# Autodesk Inventor assembly: NT_BMP005_001_A_001
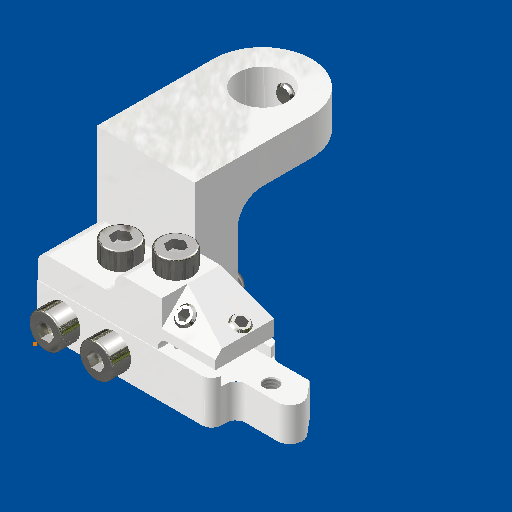
[picture p0: Inventor's stored thumbnail of the model, 512x512]
Saved by Autodesk Inventor 2025 (Build 290162000, 162)
## iProperties
Created: 2024-04-15
Part Number: NT_BMP005_001_A_001
Document SubType Name: Assembly
Designer: AdminForWorker
Mass: 69.6726 g
Surface Area: 73.8682 cm^2
Volume: 8.92251 cm^3
Density: 7.80863 g/cm^3
Title: NT_BMP005_001_A_001
Author: AdminForWorker
Revision Number: 1
## Documents named in this file (12)
- C:\Users\faricci\Inventor\Headframe_Edit\2_screws\Fabio_edit_2Screws.iam
- C:\Users\faricci\Inventor\Headframe_Edit\2_screws\Base.ipt
- C:\Users\faricci\Inventor\Headframe_Edit\2_screws\Top Base.ipt
- C:\Users\faricci\Inventor\Headframe_Edit\2_screws\Headpost_mirrored_2screws v5.ipt
- C:\Users\faricci\Inventor\Headframe_Edit\2_screws\Stereotaxic_mounting.ipt
- C:\Users\faricci\OneDrive - Fondazione Istituto Italiano Tecnologia\Documents\Inventor\Content Center Files\R2025\en-US\ISO 4026\ISO 4026 - M3 x 5 - ISO.ipt
- C:\Users\faricci\OneDrive - Fondazione Istituto Italiano Tecnologia\Documents\Inventor\Content Center Files\R2025\en-US\ISO 4026\ISO 4026 - M3 x 8 - ISO.ipt
- C:\Users\faricci\OneDrive - Fondazione Istituto Italiano Tecnologia\Documents\Inventor\Content Center Files\R2025\en-US\ISO 4762(2)\ISO 4762 - M3 x 5ISO.ipt
- C:\Users\faricci\OneDrive - Fondazione Istituto Italiano Tecnologia\Documents\Inventor\Content Center Files\R2025\en-US\ISO 4762(2)\ISO 4762 - M3 x 16ISO.ipt
- C:\Users\faricci\OneDrive - Fondazione Istituto Italiano Tecnologia\Documents\Inventor\Content Center Files\R2025\en-US\ISO 4762(2)\ISO 4762 - M3 x 12ISO.ipt
- C:\Users\faricci\OneDrive - Fondazione Istituto Italiano Tecnologia\Documents\Inventor\Content Center Files\R2025\en-US\ISO 4762(2)\ISO 4762 - M3 x 20ISO.ipt
- C:\Users\faricci\OneDrive - Fondazione Istituto Italiano Tecnologia\Documents\Inventor\Content Center Files\R2025\en-US\ISO 4032(2)\ISO 4032 - M2.5 - ISO.ipt
## Components (14 placed, 11 different names)
1. 0160-300-10(Mirror):1 — Rigid:1, Rigid:2, Rigid:3, Mate:3, Mate:6, Mate:7, Mate:8, Mate:9
2. 0160-300-01 (Mirror):1 — Rigid:2, Mate:1, Mate:2, Insert:1, Insert:2
3. Headpost_mirrored_2screws v5:1 — Rigid:3, Mate:4
4. Stereotaxic_mounting:2 — Rigid:1, Mate:5, Insert:3, Insert:4
5. ISO 4026 M3 x 5:1 — Mate:1
6. ISO 4026 M3 x 8:1 — Mate:2
7. ISO 4762 M3 x 5:1 — Mate:3, Mate:4
8. ISO 4762 M3 x 16:1 — Insert:1
9. ISO 4762 M3 x 12:1 — Insert:2
10. ISO 4026 M3 x 5:2 — Mate:5
11. ISO 4762 M3 x 20:1 — Mate:6, Mate:7
12. ISO 4762 M3 x 20:2 — Mate:8, Mate:9
13. ISO 4032 M2.5:1 — Insert:3
14. ISO 4032 M2.5:2 — Insert:4
## Relationships (16: Mate 9, Insert 4, WeldJoint 3)
- Rigid:1 [WeldJoint]: 0160-300-10(Mirror):1 ↔ Stereotaxic_mounting:2
- Rigid:2 [WeldJoint]: 0160-300-10(Mirror):1 ↔ 0160-300-01 (Mirror):1
- Rigid:3 [WeldJoint]: 0160-300-10(Mirror):1 ↔ Headpost_mirrored_2screws v5:1
- Mate:1: 0160-300-01 (Mirror):1 ↔ ISO 4026 M3 x 5:1
- Mate:2: 0160-300-01 (Mirror):1 ↔ ISO 4026 M3 x 8:1
- Mate:3: 0160-300-10(Mirror):1 ↔ ISO 4762 M3 x 5:1
- Mate:4: Headpost_mirrored_2screws v5:1 ↔ ISO 4762 M3 x 5:1
- Insert:1: 0160-300-01 (Mirror):1 ↔ ISO 4762 M3 x 16:1
- Insert:2: 0160-300-01 (Mirror):1 ↔ ISO 4762 M3 x 12:1
- Mate:5: Stereotaxic_mounting:2 ↔ ISO 4026 M3 x 5:2
- Mate:6: 0160-300-10(Mirror):1 ↔ ISO 4762 M3 x 20:1
- Mate:7: 0160-300-10(Mirror):1 ↔ ISO 4762 M3 x 20:1
- Mate:8: 0160-300-10(Mirror):1 ↔ ISO 4762 M3 x 20:2
- Mate:9: 0160-300-10(Mirror):1 ↔ ISO 4762 M3 x 20:2
- Insert:3: Stereotaxic_mounting:2 ↔ ISO 4032 M2.5:1
- Insert:4: Stereotaxic_mounting:2 ↔ ISO 4032 M2.5:2
